# Autodesk Inventor assembly: GearboxShifter
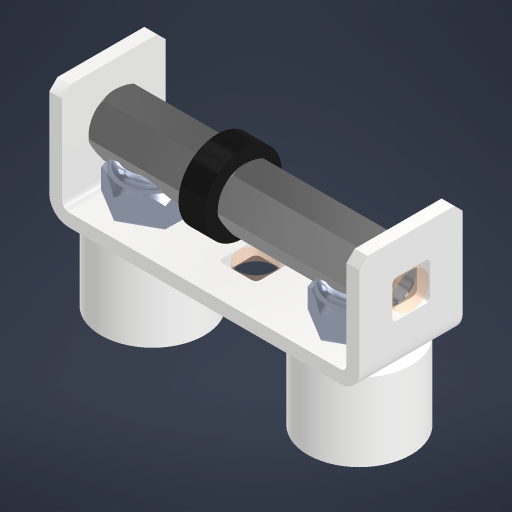
[picture p0: Inventor's stored thumbnail of the model, 512x512]
Saved by Autodesk Inventor 2023 (Build 270158000, 158)
## iProperties
Created: 2023-05-22
Part Number: GearboxShifter
Document SubType Name: Assembly
Designer: alex
Author: alex
## Documents named in this file (12)
- C:\Users\alex\Documents\GitHub\4067X-Over-Under-CAD\Chassis\GearboxShifter.iam
- C:\Users\alex\Documents\GitHub\4067X-Over-Under-CAD\VEX-CAD-Inventor\Structure\C Channel\Aluminum 1x3x1\Alu C 1x3x1x1.ipt
- C:\Users\alex\Documents\GitHub\4067X-Over-Under-CAD\VEX-CAD-Inventor\Structure\Standoff\Standoff .75.ipt
- C:\Users\alex\Documents\GitHub\4067X-Over-Under-CAD\VEX-CAD-Inventor\Structure\Standoff.ipt
- C:\Users\alex\Documents\GitHub\4067X-Over-Under-CAD\VEX-CAD-Inventor\Structure\Standoff\Standoff .50.ipt
- C:\Users\alex\Documents\GitHub\4067X-Over-Under-CAD\VEX-CAD-Inventor\Motion\Spacers\Spacer Nylon .375 OD\NSpacer .375 OD x .125.ipt
- C:\Users\alex\Documents\GitHub\4067X-Over-Under-CAD\VEX-CAD-Inventor\Motion\Spacers\Spacer Nylon .375 OD.ipt
- C:\Users\alex\Documents\GitHub\4067X-Over-Under-CAD\VEX-CAD-Inventor\Structure\Hardware\Nut Thin Nylock.ipt
- C:\Users\alex\Documents\GitHub\4067X-Over-Under-CAD\VEX-CAD-Inventor\Motion\Spacers\Spacer Nylon .500 OD\NSpacer White .500 OD x .375.ipt
- C:\Users\alex\Documents\GitHub\4067X-Over-Under-CAD\VEX-CAD-Inventor\Motion\Spacers\Spacer Nylon .500 OD.ipt
- C:\Users\alex\Documents\GitHub\4067X-Over-Under-CAD\VEX-CAD-Inventor\Structure\Hardware\Screw Steel - Star.ipt
- C:\Users\alex\Documents\GitHub\4067X-Over-Under-CAD\VEX-CAD-Inventor\Structure\Hardware\Screw Steel - Star\SScrew Star Smooth .500.ipt
## Components (10 placed, 7 different names)
1. Alu C 1x3x1x1:1 — Insert:1, Insert:2, Angle:1, Angle:2, Insert:4, Insert:5, Insert:6, Insert:7
2. Standoff .75:1 — Insert:1, Insert:3, Angle:1
3. Standoff .50:2 — Insert:2, Angle:2
4. NSpacer .375 OD x .125:1 — Insert:3
5. Nut Thin Nylock:1 — Insert:4
6. Nut Thin Nylock:2 — Insert:5
7. NSpacer White .500 OD x .375:1 — Insert:6, Insert:8
8. NSpacer White .500 OD x .375:2 — Insert:7, Insert:9
9. SScrew Star Smooth .500:1 — Insert:8
10. SScrew Star Smooth .500:2 — Insert:9
## Relationships (11: Insert 9, Angle 2)
- Insert:1: Alu C 1x3x1x1:1 ↔ Standoff .75:1
- Insert:2: Alu C 1x3x1x1:1 ↔ Standoff .50:2
- Insert:3: Standoff .75:1 ↔ NSpacer .375 OD x .125:1
- Angle:1 (0 deg): Alu C 1x3x1x1:1 ↔ Standoff .75:1
- Angle:2 (0 deg): Alu C 1x3x1x1:1 ↔ Standoff .50:2
- Insert:4: Alu C 1x3x1x1:1 ↔ Nut Thin Nylock:1
- Insert:5: Alu C 1x3x1x1:1 ↔ Nut Thin Nylock:2
- Insert:6: Alu C 1x3x1x1:1 ↔ NSpacer White .500 OD x .375:1
- Insert:7: Alu C 1x3x1x1:1 ↔ NSpacer White .500 OD x .375:2
- Insert:8 (-1.651 mm): NSpacer White .500 OD x .375:1 ↔ SScrew Star Smooth .500:1
- Insert:9 (-1.651 mm): NSpacer White .500 OD x .375:2 ↔ SScrew Star Smooth .500:2
